# Autodesk Inventor assembly: A_GERMI01-01
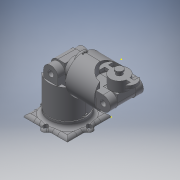
[picture p0: Inventor's stored thumbnail of the model, 180x180]
Saved by Autodesk Inventor 2016 (Build 200138000, 138)
## iProperties
Created: 2016-11-08
Part Number: A_GERMI01-01
Document SubType Name: Assembly
Designer: Kai
Author: Kai
## Documents named in this file (4)
- X:\GERMI\Project--Germi\A_GERMI01-01.iam
- X:\GERMI\Project--Germi\GERMI01-01-01.ipt
- X:\GERMI\Project--Germi\GERMI01-02-01.ipt
- X:\GERMI\Project--Germi\Germi01-03-01.ipt
## Components (7 placed, 3 different names)
1. GERMI01-01-01:1 — Insert:1
2. GERMI01-02-01:1 — Mate:1
3. GERMI01-02-01:2 — Insert:1, Mate:1, Mate:2
4. Germi01-03-01:1 — Mate:2, Insert:2
5. GERMI01-02-01:3 — Insert:2, Mate:3, Insert:3
6. GERMI01-02-01:4 — Mate:3
7. Germi01-03-01:2 — Insert:3
## Relationships (6: Insert 3, Mate 3)
- Insert:1: GERMI01-01-01:1 ↔ GERMI01-02-01:2
- Mate:1: GERMI01-02-01:1 ↔ GERMI01-02-01:2
- Mate:2: GERMI01-02-01:2 ↔ Germi01-03-01:1
- Insert:2: Germi01-03-01:1 ↔ GERMI01-02-01:3
- Mate:3: GERMI01-02-01:3 ↔ GERMI01-02-01:4
- Insert:3: GERMI01-02-01:3 ↔ Germi01-03-01:2
